# Autodesk Inventor assembly: X-Ray Tube Assy.ipt
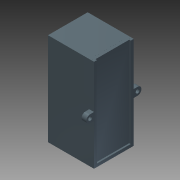
[picture p0: Inventor's stored thumbnail of the model, 180x180]
Saved by Autodesk Inventor 2015 (Build 190159000, 159)
## iProperties
Created: 2015-03-09
Part Number: X-Ray Tube Assy.ipt
Document SubType Name: Assembly
Designer: pltwe4
Author: pltwe4
## Documents named in this file (8)
- C:\Users\pltwe4\Documents\model\X-Ray Tube Assy.ipt.iam
- C:\Users\pltwe4\Documents\model\X-Ray Tube Pins.ipt
- C:\Users\pltwe4\Documents\model\X-Ray Tube.ipt
- C:\Users\pltwe4\Documents\model\X-Ray Tube End.ipt
- C:\Users\pltwe4\Documents\model\X-Ray Tube Output.ipt
- C:\Users\pltwe4\Documents\model\X-Ray Tube Plug.ipt
- C:\Users\pltwe4\Documents\model\Lead Box Cover.ipt
- C:\Users\pltwe4\Documents\model\Lead Box.ipt
## Components (12 placed, 7 different names)
1. X-Ray Tube Pins:1 — Flush:2, Mate:3, Mate:4
2. X-Ray Tube:1 — Mate:1, Mate:2, Flush:1, Mate:3, Mate:4, Mate:5, Mate:6, Mate:7, Mate:8, Mate:9, Mate:10, Flush:7, Mate:11, Mate:12, Mate:13, Mate:14
3. X-Ray Tube Pins:2 — Flush:5, Flush:6, Mate:7
4. X-Ray Tube Pins:3 — Flush:4, Flush:5, Mate:8
5. X-Ray Tube Pins:4 — Flush:2, Flush:3, Mate:9
6. X-Ray Tube Pins:5 — Flush:3, Flush:4, Mate:6
7. X-Ray Tube Pins:6 — Flush:6, Mate:5
8. X-Ray Tube End:1 — Mate:10, Flush:7
9. X-Ray Tube Output:1 — Mate:11, Mate:12, Mate:15, Mate:16, Mate:17
10. X-Ray Tube Plug:1 — Mate:13, Mate:14
11. Lead Box Cover:1 — Mate:19, Mate:20, Mate:21
12. Lead Box:1 — Mate:15, Mate:16, Mate:17, Mate:18, Mate:19, Mate:20, Mate:21
## Relationships (28: Mate 21, Flush 7)
- Mate:1: X-Ray Tube:1
- Mate:2: X-Ray Tube:1
- Flush:1: X-Ray Tube:1
- Flush:2: X-Ray Tube Pins:1 ↔ X-Ray Tube Pins:4
- Flush:3: X-Ray Tube Pins:4 ↔ X-Ray Tube Pins:5
- Flush:4: X-Ray Tube Pins:3 ↔ X-Ray Tube Pins:5
- Flush:5: X-Ray Tube Pins:2 ↔ X-Ray Tube Pins:3
- Flush:6: X-Ray Tube Pins:2 ↔ X-Ray Tube Pins:6
- Mate:3: X-Ray Tube Pins:1 ↔ X-Ray Tube:1
- Mate:4: X-Ray Tube Pins:1 ↔ X-Ray Tube:1
- Mate:5: X-Ray Tube:1 ↔ X-Ray Tube Pins:6
- Mate:6: X-Ray Tube:1 ↔ X-Ray Tube Pins:5
- Mate:7: X-Ray Tube:1 ↔ X-Ray Tube Pins:2
- Mate:8: X-Ray Tube:1 ↔ X-Ray Tube Pins:3
- Mate:9: X-Ray Tube:1 ↔ X-Ray Tube Pins:4
- Mate:10: X-Ray Tube:1 ↔ X-Ray Tube End:1
- Flush:7: X-Ray Tube:1 ↔ X-Ray Tube End:1
- Mate:11: X-Ray Tube:1 ↔ X-Ray Tube Output:1
- Mate:12: X-Ray Tube:1 ↔ X-Ray Tube Output:1
- Mate:13: X-Ray Tube:1 ↔ X-Ray Tube Plug:1
- Mate:14: X-Ray Tube:1 ↔ X-Ray Tube Plug:1
- Mate:15: X-Ray Tube Output:1 ↔ Lead Box:1
- Mate:16: X-Ray Tube Output:1 ↔ Lead Box:1
- Mate:17: X-Ray Tube Output:1 ↔ Lead Box:1
- Mate:18: Lead Box:1
- Mate:19: Lead Box Cover:1 ↔ Lead Box:1
- Mate:20: Lead Box Cover:1 ↔ Lead Box:1
- Mate:21: Lead Box Cover:1 ↔ Lead Box:1
